# Autodesk Inventor assembly: LARDIS_1
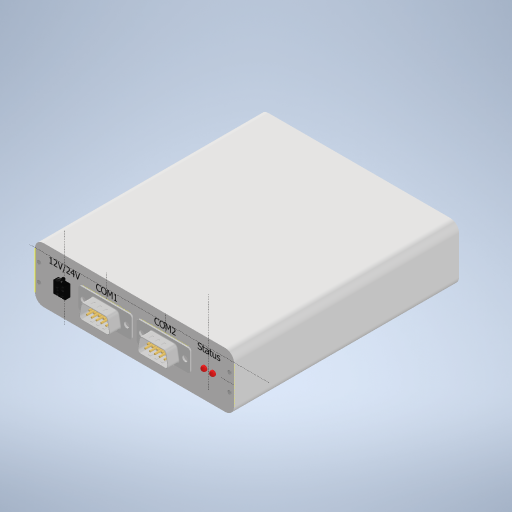
[picture p0: Inventor's stored thumbnail of the model, 512x512]
Saved by Autodesk Inventor 2024.2 (Build 282272000, 272)
## iProperties
Created: 2024-04-17
Part Number: LARDIS_1
Document SubType Name: Assembly
Designer: Holger
Author: Holger
## iProperties of the stored document 203632-0401.ipt
Created: 2019-06-19
Part Number: 2036320401
Material: Generisch
Document SubType Name: Modeling
Designer: Holger
Density: 1 g/cm^3
Appearance: Vorgabe
Sending System: PRO/ENGINEER BY PARAMETRIC TECHNOLOGY CORPORATION, 2016010
Preprocessor: PRO/ENGINEER BY PARAMETRIC TECHNOLOGY CORPORATION, 2016010
Title: 2036320401
Author: gga
Revision Number: 3LAST_VERSION
## Documents named in this file (6)
- C:\Users\holge\Desktop\19inch LARDIS\LARDIS_Box.iam
- C:\Users\holge\Desktop\19inch LARDIS\Lardis_grob.ipt
- C:\Users\holge\Desktop\19inch LARDIS\subd9\1216770.iam
- **C:\Users\holge\Desktop\19inch LARDIS\LARDIS_Box.iam*LocalDocs*xAaaaqddaAaaaaaaaAaaaa2ttGb*203632-0401.ipt
- C:\Users\holge\Desktop\19inch LARDIS\extern\LED 3mm\sli-343yc3f_03.ipt
- C:\Users\holge\Desktop\19inch LARDIS\extern\203632-0401.stp
## Components (6 placed, 4 different names)
1. Lardis_grob:1 — Fluchtend:1, Fluchtend:2, Passend:1, Passend:2, Passend:3, Fluchtend:5, Passend:7, Passend:5, Passend:6, Fluchtend:6, Passend:8, Fluchtend:7, Fluchtend:8, Fluchtend:9, Passend:9, Passend:10, Fluchtend:10, Fluchtend:11
2. 1216770:1 [sub-assembly] — Fluchtend:1, Passend:5, Passend:6
3. 1216770:2 [sub-assembly] — Fluchtend:2, Fluchtend:5, Passend:7
4. 203632-0401:1 — Fluchtend:6, Passend:8, Fluchtend:7
5. sli-343yc3f_03:1 — Fluchtend:8, Passend:9, Fluchtend:11
6. sli-343yc3f_03:2 — Fluchtend:9, Passend:10, Fluchtend:10
## Relationships (18: Flush 9, Mate 9)
- Fluchtend:1 [Flush] (-1 mm): Lardis_grob:1 ↔ 1216770:1
- Fluchtend:2 [Flush] (-1 mm): Lardis_grob:1 ↔ 1216770:2
- Passend:1 [Mate]: Lardis_grob:1
- Passend:2 [Mate]: Lardis_grob:1
- Passend:3 [Mate]: Lardis_grob:1
- Fluchtend:5 [Flush] (39.8 mm): Lardis_grob:1 ↔ 1216770:2
- Passend:7 [Mate] (-16 mm): Lardis_grob:1 ↔ 1216770:2
- Passend:5 [Mate] (-16 mm): Lardis_grob:1 ↔ 1216770:1
- Passend:6 [Mate] (-41.5 mm): Lardis_grob:1 ↔ 1216770:1
- Fluchtend:6 [Flush] (-3 mm): Lardis_grob:1 ↔ 203632-0401:1
- Passend:8 [Mate] (-17 mm): Lardis_grob:1 ↔ 203632-0401:1
- Fluchtend:7 [Flush] (16 mm): Lardis_grob:1 ↔ 203632-0401:1
- Fluchtend:8 [Flush] (0.1 mm): Lardis_grob:1 ↔ sli-343yc3f_03:1
- Fluchtend:9 [Flush] (0.1 mm): Lardis_grob:1 ↔ sli-343yc3f_03:2
- Passend:9 [Mate] (-16 mm): Lardis_grob:1 ↔ sli-343yc3f_03:1
- Passend:10 [Mate] (-16 mm): Lardis_grob:1 ↔ sli-343yc3f_03:2
- Fluchtend:10 [Flush] (12 mm): Lardis_grob:1 ↔ sli-343yc3f_03:2
- Fluchtend:11 [Flush] (17 mm): Lardis_grob:1 ↔ sli-343yc3f_03:1
